# Autodesk Inventor assembly: Quick Assembly
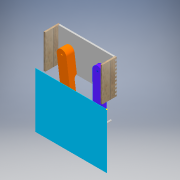
[picture p0: Inventor's stored thumbnail of the model, 180x180]
Saved by Autodesk Inventor 2017 (Build 210142000, 142)
## iProperties
Created: 2017-04-26
Part Number: Quick Assembly
Document SubType Name: Assembly
Designer: Parshant Bombhi
Author: Parshant Bombhi
## Documents named in this file (11)
- C:\Users\Parshant Bombhi\sfuvault\Rembrant Robotics\Parshant Files\Assembly.iam
- C:\Users\Parshant Bombhi\sfuvault\Rembrant Robotics\Parshant Files\8.5 x 11 paper.ipt
- C:\Users\Parshant Bombhi\sfuvault\Rembrant Robotics\Parshant Files\Base.ipt
- C:\Users\Parshant Bombhi\sfuvault\Rembrant Robotics\Parshant Files\Inner Arm Thin.ipt
- C:\Users\Parshant Bombhi\sfuvault\Rembrant Robotics\Parshant Files\Inner Arm Thick.ipt
- C:\Users\Parshant Bombhi\sfuvault\Rembrant Robotics\Parshant Files\Outer Arm.ipt
- C:\Users\Parshant Bombhi\sfuvault\Rembrant Robotics\Parshant Files\5-16in Shaft.ipt
- C:\Users\Parshant Bombhi\sfuvault\Rembrant Robotics\Parshant Files\5-8in clevis pin   92390A213.ipt
- C:\Users\Parshant Bombhi\sfuvault\Rembrant Robotics\Parshant Files\Cotter Pin.ipt
- C:\Users\Parshant Bombhi\sfuvault\Rembrant Robotics\Parshant Files\Pencil\pencil_assembly.iam
- C:\Users\Parshant Bombhi\sfuvault\Rembrant Robotics\Parshant Files\Side Support.ipt
## Components (15 placed, 10 different names)
1. 8.5 x 11 paper:1 — Mate:45, Mate:46, Flush:1
2. Base:1 — Mate:45, Mate:46, Flush:1, Mate:47, Mate:48, Mate:49, Mate:50, Flush:2, Flush:3, Flush:4, Mate:51, Flush:5, Flush:6
3. Inner Arm Thin:1 — Mate:20, Mate:21, Mate:29, Mate:30, Mate:31, Mate:35, Mate:36, Mate:50
4. Inner Arm Thick:1 — Mate:22, Mate:23, Mate:32, Mate:33, Mate:34, Mate:37, Mate:38, Mate:49
5. Outer Arm:1 — Mate:20, Mate:21, Mate:24
6. Outer Arm:2 — Mate:22, Mate:23, Mate:24, Mate:43, Mate:44
7. 5-16in Shaft:1 — Mate:29, Mate:30, Mate:31, Mate:47
8. 5-16in Shaft:2 — Mate:32, Mate:33, Mate:34, Mate:48
9. 5-8in clevis pin   92390A213:1 — Mate:35, Mate:36, Mate:39, Mate:40
10. 5-8in clevis pin   92390A213:2 — Mate:37, Mate:38, Mate:41, Mate:42
11. Cotter Pin:1 — Mate:41, Mate:42
12. Cotter Pin:2 — Mate:39, Mate:40
13. pencil_assembly:1 [sub-assembly] — Mate:43, Mate:44
14. Side Support:1 — Flush:2, Flush:3, Flush:4
15. Side Support:2 — Mate:51, Flush:5, Flush:6
## Relationships (34: Mate 28, Flush 6)
- Mate:20: Inner Arm Thin:1 ↔ Outer Arm:1
- Mate:21: Inner Arm Thin:1 ↔ Outer Arm:1
- Mate:22: Inner Arm Thick:1 ↔ Outer Arm:2
- Mate:23: Inner Arm Thick:1 ↔ Outer Arm:2
- Mate:24: Outer Arm:1 ↔ Outer Arm:2
- Mate:29: Inner Arm Thin:1 ↔ 5-16in Shaft:1
- Mate:30: Inner Arm Thin:1 ↔ 5-16in Shaft:1
- Mate:31: Inner Arm Thin:1 ↔ 5-16in Shaft:1
- Mate:32: Inner Arm Thick:1 ↔ 5-16in Shaft:2
- Mate:33: Inner Arm Thick:1 ↔ 5-16in Shaft:2
- Mate:34: Inner Arm Thick:1 ↔ 5-16in Shaft:2
- Mate:35: Inner Arm Thin:1 ↔ 5-8in clevis pin   92390A213:1
- Mate:36: Inner Arm Thin:1 ↔ 5-8in clevis pin   92390A213:1
- Mate:37: Inner Arm Thick:1 ↔ 5-8in clevis pin   92390A213:2
- Mate:38: Inner Arm Thick:1 ↔ 5-8in clevis pin   92390A213:2
- Mate:39: 5-8in clevis pin   92390A213:1 ↔ Cotter Pin:2
- Mate:40 (12.7 mm): 5-8in clevis pin   92390A213:1 ↔ Cotter Pin:2
- Mate:41: 5-8in clevis pin   92390A213:2 ↔ Cotter Pin:1
- Mate:42 (-12.7 mm): 5-8in clevis pin   92390A213:2 ↔ Cotter Pin:1
- Mate:43: Outer Arm:2 ↔ pencil_assembly:1
- Mate:44 (25.4 mm): Outer Arm:2 ↔ pencil_assembly:1
- Mate:45: 8.5 x 11 paper:1 ↔ Base:1
- Mate:46 (57.15 mm): 8.5 x 11 paper:1 ↔ Base:1
- Flush:1 (25.4 mm): 8.5 x 11 paper:1 ↔ Base:1
- Mate:47: Base:1 ↔ 5-16in Shaft:1
- Mate:48: Base:1 ↔ 5-16in Shaft:2
- Mate:49: Base:1 ↔ Inner Arm Thick:1
- Mate:50 (2.54 mm): Base:1 ↔ Inner Arm Thin:1
- Flush:2: Base:1 ↔ Side Support:1
- Flush:3: Base:1 ↔ Side Support:1
- Flush:4: Base:1 ↔ Side Support:1
- Mate:51: Base:1 ↔ Side Support:2
- Flush:5: Base:1 ↔ Side Support:2
- Flush:6: Base:1 ↔ Side Support:2
